# Autodesk Inventor assembly: Ensamblaje1
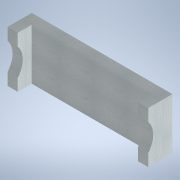
[picture p0: Inventor's stored thumbnail of the model, 180x180]
Saved by Autodesk Inventor 2022.4 (Build 264492010, 492A)
## iProperties
Created: 2023-02-14
Part Number: Ensamblaje1
Document SubType Name: Assembly
Designer: wob19
Author: wob19
## Documents named in this file (4)
- C:\Users\wob19\OneDrive - Universidad Nacional de Colombia\Materias UN\APM\Piezas\Ensamblaje1.iam
- C:\Users\wob19\OneDrive - Universidad Nacional de Colombia\Materias UN\APM\Piezas\soporte.ipt
- C:\Users\wob19\OneDrive - Universidad Nacional de Colombia\Materias UN\APM\Piezas\Base.ipt
- C:\Users\wob19\OneDrive - Universidad Nacional de Colombia\Materias UN\APM\Piezas\union.ipt
## Components (7 placed, 3 different names)
1. soporte:1 — Insertar:3, Insertar:4
2. soporte:2 — Insertar:1, Insertar:2
3. Base:1 — Rígido:1, Rígido:2, Rígido:3, Rígido:4
4. union:1 — Rígido:1, Insertar:4
5. union:2 — Rígido:2, Insertar:1
6. union:3 — Rígido:3, Insertar:2
7. union:4 — Rígido:4, Insertar:3
## Relationships (8: WeldJoint 4, Insert 4)
- Rígido:1 [WeldJoint]: Base:1 ↔ union:1
- Rígido:2 [WeldJoint]: Base:1 ↔ union:2
- Rígido:3 [WeldJoint]: Base:1 ↔ union:3
- Rígido:4 [WeldJoint]: Base:1 ↔ union:4
- Insertar:1 (-13 mm): soporte:2 ↔ union:2
- Insertar:2 (-13 mm): soporte:2 ↔ union:3
- Insertar:3 (-13 mm): soporte:1 ↔ union:4
- Insertar:4 (-13 mm): soporte:1 ↔ union:1
